# Autodesk Inventor assembly: Front fixed top coupler assembly
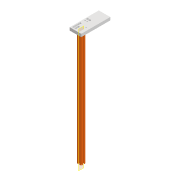
[picture p0: Inventor's stored thumbnail of the model, 180x180]
Saved by Autodesk Inventor 2020 (Build 240168000, 168)
## iProperties
Created: 2019-11-14
Part Number: Front fixed top coupler assembly
Document SubType Name: Assembly
Designer: ball
Author: ball
## Documents named in this file (3)
- C:\FTC\FTC8863CAD\2019 Robot\Delivery\Front fixed top coupler assembly.iam
- C:\FTC\FTC8863CAD\2019 Robot\Delivery\Fixed top coupler.ipt
- C:\FTC\FTC8863CAD\RevRobotics\REV-41-1017_15mm_extrusion_17.875in.ipt
## Components (2 placed, 2 different names)
1. Fixed top coupler:1 — Mate:1, Flush:1, Flush:2
2. REV-41-1017_15mm_extrusion_17.875in:1 — Mate:1, Flush:1, Flush:2
## Relationships (3: Flush 2, Mate 1)
- Mate:1: Fixed top coupler:1 ↔ REV-41-1017_15mm_extrusion_17.875in:1
- Flush:1 (1.27 mm): Fixed top coupler:1 ↔ REV-41-1017_15mm_extrusion_17.875in:1
- Flush:2 (1.27 mm): Fixed top coupler:1 ↔ REV-41-1017_15mm_extrusion_17.875in:1
